# Autodesk Inventor assembly: collector rotator assembly
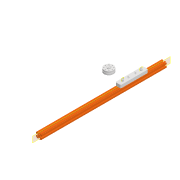
[picture p0: Inventor's stored thumbnail of the model, 180x180]
Saved by Autodesk Inventor 2020 (Build 240168000, 168)
## iProperties
Created: 2019-11-06
Part Number: collector rotator assembly
Document SubType Name: Assembly
Designer: ball
Author: ball
## Documents named in this file (7)
- C:\FTC\FTC8863CAD\2019 Robot\Collection\collector rotator assembly.iam
- C:\FTC\FTC8863CAD\2019 Robot\Collection\Collection rotation adapter.ipt
- C:\FTC\FTC8863CAD\2019 Robot\Collection\6-32x5-16.ipt
- C:\FTC\FTC8863CAD\RevRobotics\REV-41-1017_15mm_extrusion_17.875in.ipt
- C:\FTC\FTC8863CAD\StepLibraries\Screws\m3x15-8 STAINLESS STEEL HEX HEAD CAP SCREW.ipt
- C:\FTC\FTC8863CAD\StepLibraries\Nuts\m3 18-8 STAINLESS STL NYLON-INSERT LOCKNUT.ipt
- C:\FTC\FTC8863CAD\Actobotics\545 parts\545364 assembly.ipt
## Components (9 placed, 6 different names)
1. Collection rotation adapter:1 — Mate:1, Mate:2, Mate:3, Mate:4, Mate:9, Flush:1, Flush:2, Mate:10, Mate:11, Mate:12, Mate:14
2. 6-32x5-16:1 — Mate:3, Mate:4
3. 6-32x5-16:2 — Mate:1, Mate:2
4. REV-41-1017_15mm_extrusion_17.875in:1 — Mate:5, Mate:6, Mate:7, Mate:8, Mate:9, Flush:1, Flush:2
5. m3x15-8 STAINLESS STEEL HEX HEAD CAP SCREW:1 — Mate:5, Mate:6, Mate:11, Mate:13
6. m3x15-8 STAINLESS STEEL HEX HEAD CAP SCREW:2 — Mate:7, Mate:8, Mate:10, Mate:15
7. m3 18-8 STAINLESS STL NYLON-INSERT LOCKNUT:1 — Mate:12, Mate:13
8. m3 18-8 STAINLESS STL NYLON-INSERT LOCKNUT:2 — Mate:14, Mate:15
9. 545364 assembly:1
## Relationships (17: Mate 15, Flush 2)
- Mate:1: Collection rotation adapter:1 ↔ 6-32x5-16:2
- Mate:2: Collection rotation adapter:1 ↔ 6-32x5-16:2
- Mate:3: Collection rotation adapter:1 ↔ 6-32x5-16:1
- Mate:4: Collection rotation adapter:1 ↔ 6-32x5-16:1
- Mate:5: REV-41-1017_15mm_extrusion_17.875in:1 ↔ m3x15-8 STAINLESS STEEL HEX HEAD CAP SCREW:1
- Mate:6: REV-41-1017_15mm_extrusion_17.875in:1 ↔ m3x15-8 STAINLESS STEEL HEX HEAD CAP SCREW:1
- Mate:7: REV-41-1017_15mm_extrusion_17.875in:1 ↔ m3x15-8 STAINLESS STEEL HEX HEAD CAP SCREW:2
- Mate:8: REV-41-1017_15mm_extrusion_17.875in:1 ↔ m3x15-8 STAINLESS STEEL HEX HEAD CAP SCREW:2
- Mate:9: Collection rotation adapter:1 ↔ REV-41-1017_15mm_extrusion_17.875in:1
- Flush:1: Collection rotation adapter:1 ↔ REV-41-1017_15mm_extrusion_17.875in:1
- Flush:2 (50.8 mm): Collection rotation adapter:1 ↔ REV-41-1017_15mm_extrusion_17.875in:1
- Mate:10: Collection rotation adapter:1 ↔ m3x15-8 STAINLESS STEEL HEX HEAD CAP SCREW:2
- Mate:11: Collection rotation adapter:1 ↔ m3x15-8 STAINLESS STEEL HEX HEAD CAP SCREW:1
- Mate:12: Collection rotation adapter:1 ↔ m3 18-8 STAINLESS STL NYLON-INSERT LOCKNUT:1
- Mate:13: m3x15-8 STAINLESS STEEL HEX HEAD CAP SCREW:1 ↔ m3 18-8 STAINLESS STL NYLON-INSERT LOCKNUT:1
- Mate:14: Collection rotation adapter:1 ↔ m3 18-8 STAINLESS STL NYLON-INSERT LOCKNUT:2
- Mate:15: m3x15-8 STAINLESS STEEL HEX HEAD CAP SCREW:2 ↔ m3 18-8 STAINLESS STL NYLON-INSERT LOCKNUT:2
